# Autodesk Inventor assembly: the bot
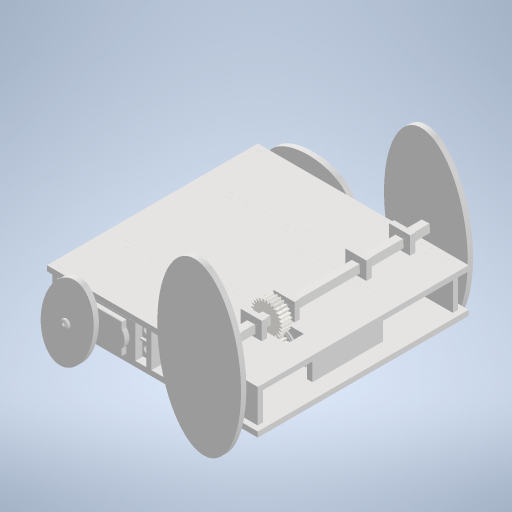
[picture p0: Inventor's stored thumbnail of the model, 512x512]
Saved by Autodesk Inventor 2023 (Build 270158000, 158)
## iProperties
Created: 2023-11-13
Part Number: the bot
Document SubType Name: Assembly
Designer: Nate
Author: Nate
## Documents named in this file (17)
- C:\Users\Nate\Desktop\Bio robot\the bot.iam
- C:\Users\Nate\Desktop\Bio robot\base.ipt
- C:\Users\Nate\Documents\CAD_Assignment_2\Servo Assembly\Servo Assembly.iam
- C:\Users\Nate\Documents\CAD_Assignment_2\McMaster-Carr imports\95836A255_Black-Oxide 18-8 Stainless Steel Pan Head Phillips Screws.ipt
- C:\Users\Nate\Desktop\Bio robot\top.ipt
- C:\Users\Nate\Desktop\Bio robot\servo long side.ipt
- C:\Users\Nate\Desktop\Bio robot\servo short side.ipt
- C:\Users\Nate\Desktop\Bio robot\servo longer short side.ipt
- C:\Users\Nate\Desktop\Bio robot\servo front.ipt
- C:\Users\Nate\Desktop\Bio robot\front support.ipt
- C:\Users\Nate\Desktop\Bio robot\rod holder.ipt
- C:\Users\Nate\Desktop\Bio robot\arms front.ipt
- C:\Users\Nate\Desktop\Bio robot\arms back.ipt
- C:\Users\Nate\Desktop\Bio robot\drive gear.ipt
- C:\Users\Nate\Desktop\Bio robot\drive shaft.ipt
- C:\Users\Nate\Desktop\Bio robot\bushings.ipt
- C:\Users\Nate\Desktop\Bio robot\top gear.ipt
## Components (38 placed, 15 different names)
1. base:1 — Flush:2, Mate:3, Mate:4, Mate:5, Mate:6, Mate:7, Mate:8, Mate:9, Mate:10, Mate:11, Mate:12, Mate:13, Mate:14, Mate:15, Mate:16, Mate:17, Mate:18, Mate:19, Mate:20, Mate:21, Mate:22, Mate:23, Mate:24, Mate:25, Mate:26, Mate:27, Mate:28, Mate:29, Mate:31, Mate:32, Mate:34
2. Servo Assembly:1 [sub-assembly] — Mate:28, Mate:29, Mate:30, Mate:56
3. Servo Assembly:2 [sub-assembly] — Mate:31, Mate:32, Mate:33, Mate:55
4. Servo Assembly:3 [sub-assembly] — Mate:34, Mate:35, Mate:36, Rotational:1
5. 95836A255_Black-Oxide 18-8 Stainless Steel Pan Head Phillips Screws:1
6. top:1 — Mate:37, Mate:38, Mate:41, Mate:42, Mate:43, Mate:44, Mate:45, Mate:46, Mate:47, Mate:48, Mate:49, Mate:50
7. servo long side:1 — Flush:2, Mate:3, Mate:4
8. servo short side:1 — Mate:5, Mate:6
9. servo long side:2 — Mate:9, Mate:10
10. servo long side:3 — Mate:15, Mate:16, Mate:35
11. servo short side:2 — Mate:7, Mate:8, Mate:30
12. servo short side:3 — Mate:13, Mate:14
13. servo short side:4 — Mate:11, Mate:12, Mate:33
14. servo longer short side:1 — Mate:17, Mate:18, Mate:19, Mate:36, Mate:37, Mate:38
15. servo longer short side:2 — Mate:20, Mate:21
16. servo front:1 — Mate:22, Mate:23
17. front support:1 — Mate:24, Mate:25
18. front support:2 — Mate:26, Mate:27
19. rod holder:1 — Mate:41, Mate:42, Rotational:2
20. rod holder:2 — Mate:43, Mate:49, Rotational:3
21. rod holder:3 — Mate:44, Mate:50, Rotational:4
22. rod holder:4 — Mate:45, Mate:47, Rotational:5
23. rod holder:5 — Mate:46, Mate:48, Rotational:6
24. arms front:1 — Mate:57, Mate:58
25. arms front:2
26. arms back:1 — Mate:56, Insert:5
27. arms back:2 — Mate:55, Insert:4
28. 95836A255_Black-Oxide 18-8 Stainless Steel Pan Head Phillips Screws:2 — Insert:4
29. 95836A255_Black-Oxide 18-8 Stainless Steel Pan Head Phillips Screws:3 — Insert:5
30. Spur Gear2:1 — Rotational:1
31. drive shaft:1 — Mate:57, Mate:58
32. bushings:1 — Rotational:6
33. bushings:3 — Rotational:5
34. bushings:5 — Rotational:4
35. bushings:7 — Rotational:3
36. bushings:9 — Rotational:2
37. Spur Gear2:2 — Rigid:1
38. Spur Gear2:3 — Rigid:1
## Relationships (60: Mate 50, RevoluteJoint 6, Insert 2, Flush 1, WeldJoint 1)
- Flush:2: base:1 ↔ servo long side:1
- Mate:3: base:1 ↔ servo long side:1
- Mate:4: base:1 ↔ servo long side:1
- Mate:5: base:1 ↔ servo short side:1
- Mate:6: base:1 ↔ servo short side:1
- Mate:7: base:1 ↔ servo short side:2
- Mate:8: base:1 ↔ servo short side:2
- Mate:9: base:1 ↔ servo long side:2
- Mate:10: base:1 ↔ servo long side:2
- Mate:11: base:1 ↔ servo short side:4
- Mate:12: base:1 ↔ servo short side:4
- Mate:13: base:1 ↔ servo short side:3
- Mate:14: base:1 ↔ servo short side:3
- Mate:15: base:1 ↔ servo long side:3
- Mate:16: base:1 ↔ servo long side:3
- Mate:17: base:1 ↔ servo longer short side:1
- Mate:18: base:1 ↔ servo longer short side:1
- Mate:19: base:1 ↔ servo longer short side:1
- Mate:20: base:1 ↔ servo longer short side:2
- Mate:21: base:1 ↔ servo longer short side:2
- Mate:22: base:1 ↔ servo front:1
- Mate:23: base:1 ↔ servo front:1
- Mate:24: base:1 ↔ front support:1
- Mate:25: base:1 ↔ front support:1
- Mate:26: base:1 ↔ front support:2
- Mate:27: base:1 ↔ front support:2
- Mate:28: base:1 ↔ Servo Assembly:1
- Mate:29: base:1 ↔ Servo Assembly:1
- Mate:30 (0.5 mm): Servo Assembly:1 ↔ servo short side:2
- Mate:31: base:1 ↔ Servo Assembly:2
- Mate:32: base:1 ↔ Servo Assembly:2
- Mate:33 (0.5 mm): Servo Assembly:2 ↔ servo short side:4
- Mate:34: base:1 ↔ Servo Assembly:3
- Mate:35: Servo Assembly:3 ↔ servo long side:3
- Mate:36 (0.5 mm): Servo Assembly:3 ↔ servo longer short side:1
- Mate:37: top:1 ↔ servo longer short side:1
- Mate:38: top:1 ↔ servo longer short side:1
- Mate:41: top:1 ↔ rod holder:1
- Mate:42: top:1 ↔ rod holder:1
- Mate:43: top:1 ↔ rod holder:2
- Mate:44: top:1 ↔ rod holder:3
- Mate:45: top:1 ↔ rod holder:4
- Mate:46: top:1 ↔ rod holder:5
- Mate:47: top:1 ↔ rod holder:4
- Mate:48: top:1 ↔ rod holder:5
- Mate:49: top:1 ↔ rod holder:2
- Mate:50: top:1 ↔ rod holder:3
- Mate:55: Servo Assembly:2 ↔ arms back:2
- Insert:4: arms back:2 ↔ 95836A255_Black-Oxide 18-8 Stainless Steel Pan Head Phillips Screws:2
- Mate:56: Servo Assembly:1 ↔ arms back:1
- Insert:5: arms back:1 ↔ 95836A255_Black-Oxide 18-8 Stainless Steel Pan Head Phillips Screws:3
- Rotational:1 [RevoluteJoint]: Servo Assembly:3 ↔ Spur Gear2:1
- Rotational:2 [RevoluteJoint]: rod holder:1 ↔ bushings:9
- Rotational:3 [RevoluteJoint]: rod holder:2 ↔ bushings:7
- Rotational:4 [RevoluteJoint]: rod holder:3 ↔ bushings:5
- Rotational:5 [RevoluteJoint]: rod holder:4 ↔ bushings:3
- Rotational:6 [RevoluteJoint]: rod holder:5 ↔ bushings:1
- Mate:57: arms front:1 ↔ drive shaft:1
- Mate:58: arms front:1 ↔ drive shaft:1
- Rigid:1 [WeldJoint]: Spur Gear2:2 ↔ Spur Gear2:3
